# Autodesk Inventor assembly: Multi-Cat-mentor
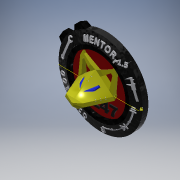
[picture p0: Inventor's stored thumbnail of the model, 180x180]
Saved by Autodesk Inventor 2017 (Build 210142000, 142)
## iProperties
Created: 2015-06-02
Part Number: Multi-Cat-mentor
Document SubType Name: Assembly
Designer: Spooner
Author: Spooner
## Documents named in this file (9)
- C:\Users\Roksbot\Documents\Inventor\Robotics Pin 2016\Multi-Cat-mentor.iam
- C:\Users\Roksbot\Documents\Inventor\Robotics Pin 2016\Background.ipt
- C:\Users\Roksbot\Documents\Inventor\Robotics Pin 2016\Disk.ipt
- C:\Users\Roksbot\Documents\Inventor\Robotics Pin 2016\Numbers.ipt
- C:\Users\Roksbot\Documents\Inventor\Robotics Pin 2016\Cat.ipt
- C:\Users\Roksbot\Documents\Inventor\Robotics Pin 2016\Eyes.ipt
- C:\Users\Roksbot\Documents\Inventor\Robotics Pin 2016\Mentor Details.ipt
- C:\Users\Roksbot\Documents\Inventor\Robotics Pin 2016\Mentor Ring.ipt
- C:\Users\Roksbot\Documents\Inventor\Robotics Pin 2016\Mentor Text.ipt
## Components (8 placed, 8 different names)
1. Background:1 — Insert:1, Angle:2, Mate:3, Mate:4, Mate:5, Mate:6
2. Disk:1 — Mate:1, Mate:2, Insert:1, Angle:1, Angle:2, Tangent:1, Angle:3, Insert:2, Angle:4
3. Numbers:1 — Mate:3, Mate:4, Mate:5
4. Cat:1 — Mate:6, Tangent:1, Angle:3, Mate:7, Mate:8, Mate:9
5. Eyes:1 — Mate:7, Mate:8, Mate:9
6. Mentor Details:1 — Insert:3, Mate:13
7. Mentor Ring:1 — Insert:2, Angle:4, Mate:10, Mate:11, Mate:12, Insert:3, Mate:13
8. Mentor Text:1 — Mate:10, Mate:11, Mate:12
## Relationships (21: Mate 13, Angle 4, Insert 3, Tangent 1)
- Mate:1: Disk:1
- Mate:2: Disk:1
- Insert:1: Background:1 ↔ Disk:1
- Angle:1 (0 deg): Disk:1
- Angle:2 (0 deg): Background:1 ↔ Disk:1
- Mate:3: Background:1 ↔ Numbers:1
- Mate:4: Background:1 ↔ Numbers:1
- Mate:5: Background:1 ↔ Numbers:1
- Mate:6: Background:1 ↔ Cat:1
- Tangent:1: Disk:1 ↔ Cat:1
- Angle:3 (0 deg): Disk:1 ↔ Cat:1
- Mate:7: Cat:1 ↔ Eyes:1
- Mate:8: Cat:1 ↔ Eyes:1
- Mate:9: Cat:1 ↔ Eyes:1
- Insert:2: Disk:1 ↔ Mentor Ring:1
- Angle:4 (180 deg): Disk:1 ↔ Mentor Ring:1
- Mate:10: Mentor Ring:1 ↔ Mentor Text:1
- Mate:11: Mentor Ring:1 ↔ Mentor Text:1
- Mate:12: Mentor Ring:1 ↔ Mentor Text:1
- Insert:3: Mentor Details:1 ↔ Mentor Ring:1
- Mate:13: Mentor Details:1 ↔ Mentor Ring:1
